# Autodesk Inventor assembly: Jetson & Carrier Board
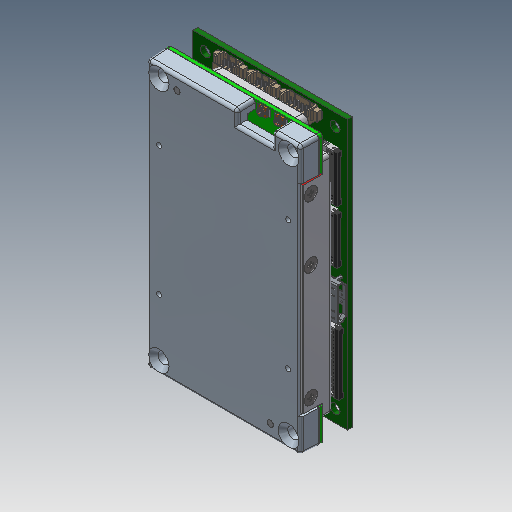
[picture p0: Inventor's stored thumbnail of the model, 512x512]
Saved by Autodesk Inventor 2019.4 (Build 234330000, 330)
## iProperties
Created: 2019-07-17
Part Number: Jetson & Carrier Board
Material: 一般
Document SubType Name: Assembly
Designer: y6tada
Author: y6tada
## Documents named in this file (4)
- C:\Workspace\Yuni8\Libs\Jetson & Carrier Board\Jetson & Carrier Board.iam
- C:\Workspace\Yuni8\Libs\Jetson & Carrier Board\Jetson TX2\jetson_tx2_with_housing.iam
- C:\Workspace\Yuni8\Libs\Jetson & Carrier Board\Auvidea J100 Carrier Board\38188-2.iam
- C:\Workspace\Yuni8\Libs\UP3-MIBV-4-CM\CUI_UP3-MIBV-4-CM.iam
## Components (3 placed, 3 different names)
1. jetson_tx2_with_housing:1 [sub-assembly] — メイト:2, メイト:3, メイト:4
2. 38188-2:1 [sub-assembly] — フラッシュ:1, フラッシュ:2, メイト:1, メイト:2, メイト:3, メイト:4, メイト:5
3. CUI_UP3-MIBV-4-CM:1 [sub-assembly] — メイト:5
## Relationships (7: Mate 5, Flush 2)
- フラッシュ:1 [Flush]: 38188-2:1
- フラッシュ:2 [Flush]: 38188-2:1
- メイト:1 [Mate]: 38188-2:1
- メイト:2 [Mate]: jetson_tx2_with_housing:1 ↔ 38188-2:1
- メイト:3 [Mate]: jetson_tx2_with_housing:1 ↔ 38188-2:1
- メイト:4 [Mate] (8 mm): jetson_tx2_with_housing:1 ↔ 38188-2:1
- メイト:5 [Mate]: 38188-2:1 ↔ CUI_UP3-MIBV-4-CM:1
